# Autodesk Inventor assembly: A_Flightcontroller_PCB
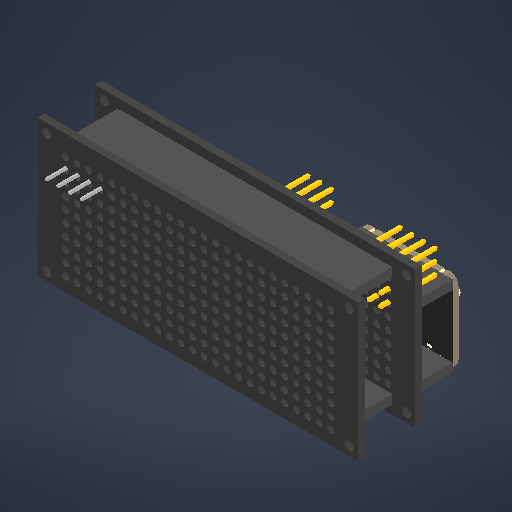
[picture p0: Inventor's stored thumbnail of the model, 512x512]
Saved by Autodesk Inventor 2026 (Build 300175000, 175)
## iProperties
Created: 2025-09-06
Part Number: A_Flightcontroller_PCB
Document SubType Name: Assembly
Designer: FAL
Author: FAL
## Documents named in this file (9)
- C:\Users\FAL\Projekte\Git\AIRBERT\CAD\Electronic\Flightcontroller_PCB\A_Flightcontroller_PCB.iam
- C:\Users\FAL\Projekte\Git\AIRBERT\CAD\Electronic\Flightcontroller_PCB\P_PCB_40x60.ipt
- C:\Users\FAL\Projekte\Git\AIRBERT\CAD\Electronic\Flightcontroller_PCB\P_Spacer_Dummy.ipt
- C:\Users\FAL\Projekte\Git\AIRBERT\CAD\Electronic\Flightcontroller_PCB\PinHeader\Pin Header 1x3 TH Pitch 2.54mm\Pin Header 1x3 TH Pitch 2.54mm\Pin Header 1x3 TH Pitch 2.54mm.ipt
- C:\Users\FAL\Projekte\Git\AIRBERT\CAD\Electronic\Flightcontroller_PCB\PinHeader\Pin Header 1x3 TH Pitch 2.54mm\AHT20+BMP280\AHT20+BMP280.ipt
- C:\Users\FAL\Projekte\Git\AIRBERT\CAD\Electronic\Flightcontroller_PCB\PinHeader\Pin Header 1x3 TH Pitch 2.54mm\MPU6050 Accelerometer\MPU6050 Accelerometer.ipt
- C:\Users\FAL\Projekte\Git\AIRBERT\CAD\Electronic\Flightcontroller_PCB\XIAO-ESP32S3 v2.iam
- C:\Users\FAL\Projekte\Git\AIRBERT\CAD\Electronic\Flightcontroller_PCB\P_Spacer_Dummy_ESP32C3.ipt
- C:\Users\FAL\Projekte\Git\AIRBERT\CAD\Electronic\Flightcontroller_PCB\resistors\Resistor Axial 0.5W - Pitch 12.7mm (500mil) - Value 270R\Resistor Axial 0.5W - Pitch 12.7mm (500mil) - Value 270R\Resistor Axial 0.ipt
## Components (19 placed, 8 different names)
1. P_PCB_40x60:1 — Fluchtend:1, Fluchtend:2, Fluchtend:5, Fluchtend:6, Fluchtend:7, Passend:2, Fluchtend:15, Passend:4, Passend:12, Passend:13
2. P_PCB_40x60:2 — Fluchtend:3, Fluchtend:4, Passend:3, Passend:8, Passend:9, Passend:10, Passend:11, Passend:15
3. P_Spacer_Dummy:1 — Passend:2, Passend:3, Fluchtend:13, Fluchtend:14
4. P_Spacer_Dummy:3 — Fluchtend:14, Fluchtend:15, Passend:4, Fluchtend:18
5. Pin Header 1x3 TH Pitch 2.54mm:1 — Passend:11
6. Pin Header 1x3 TH Pitch 2.54mm:2 — Passend:10
7. Pin Header 1x3 TH Pitch 2.54mm:3 — Passend:9
8. Pin Header 1x3 TH Pitch 2.54mm:4 — Passend:8
9. AHT20+BMP280:1 — Passend:12
10. MPU6050 Accelerometer:1 — Passend:13
11. XIAO-ESP32S3 v2:1 [sub-assembly] — Fluchtend:16, Fluchtend:17, Passend:16, Passend:17, Fluchtend:20
12. P_Spacer_Dummy_ESP32C3:1 — Passend:15, Fluchtend:16, Fluchtend:17, Passend:16, Fluchtend:18, Fluchtend:19
13. P_Spacer_Dummy_ESP32C3:2 — Fluchtend:19, Passend:17, Fluchtend:20
14. Pin Header 1x3 TH Pitch 2.54mm:9
15. Pin Header 1x3 TH Pitch 2.54mm:10
16. Pin Header 1x3 TH Pitch 2.54mm:12
17. Resistor Axial 0:1
18. Resistor Axial 0:2
19. Resistor Axial 0:3
## Relationships (27: Flush 15, Mate 12)
- Fluchtend:1 [Flush]: P_PCB_40x60:1
- Fluchtend:2 [Flush]: P_PCB_40x60:1
- Fluchtend:3 [Flush]: P_PCB_40x60:2
- Fluchtend:4 [Flush]: P_PCB_40x60:2
- Fluchtend:5 [Flush]: P_PCB_40x60:1
- Fluchtend:6 [Flush]: P_PCB_40x60:1
- Fluchtend:7 [Flush]: P_PCB_40x60:1
- Passend:2 [Mate]: P_PCB_40x60:1 ↔ P_Spacer_Dummy:1
- Passend:3 [Mate]: P_PCB_40x60:2 ↔ P_Spacer_Dummy:1
- Fluchtend:13 [Flush]: P_Spacer_Dummy:1
- Fluchtend:14 [Flush]: P_Spacer_Dummy:1 ↔ P_Spacer_Dummy:3
- Fluchtend:15 [Flush] (2 mm): P_PCB_40x60:1 ↔ P_Spacer_Dummy:3
- Passend:4 [Mate]: P_PCB_40x60:1 ↔ P_Spacer_Dummy:3
- Passend:8 [Mate]: P_PCB_40x60:2 ↔ Pin Header 1x3 TH Pitch 2.54mm:4
- Passend:9 [Mate]: P_PCB_40x60:2 ↔ Pin Header 1x3 TH Pitch 2.54mm:3
- Passend:10 [Mate]: P_PCB_40x60:2 ↔ Pin Header 1x3 TH Pitch 2.54mm:2
- Passend:11 [Mate]: P_PCB_40x60:2 ↔ Pin Header 1x3 TH Pitch 2.54mm:1
- Passend:12 [Mate]: P_PCB_40x60:1 ↔ AHT20+BMP280:1
- Passend:13 [Mate]: P_PCB_40x60:1 ↔ MPU6050 Accelerometer:1
- Passend:15 [Mate]: P_PCB_40x60:2 ↔ P_Spacer_Dummy_ESP32C3:1
- Fluchtend:16 [Flush]: XIAO-ESP32S3 v2:1 ↔ P_Spacer_Dummy_ESP32C3:1
- Fluchtend:17 [Flush]: XIAO-ESP32S3 v2:1 ↔ P_Spacer_Dummy_ESP32C3:1
- Passend:16 [Mate]: XIAO-ESP32S3 v2:1 ↔ P_Spacer_Dummy_ESP32C3:1
- Fluchtend:18 [Flush]: P_Spacer_Dummy:3 ↔ P_Spacer_Dummy_ESP32C3:1
- Fluchtend:19 [Flush]: P_Spacer_Dummy_ESP32C3:1 ↔ P_Spacer_Dummy_ESP32C3:2
- Passend:17 [Mate]: XIAO-ESP32S3 v2:1 ↔ P_Spacer_Dummy_ESP32C3:2
- Fluchtend:20 [Flush]: XIAO-ESP32S3 v2:1 ↔ P_Spacer_Dummy_ESP32C3:2
